# Autodesk Inventor assembly: Sostenedor puerta caja
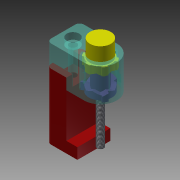
[picture p0: Inventor's stored thumbnail of the model, 180x180]
Saved by Autodesk Inventor 2014 (Build 180170000, 170)
## iProperties
Created: 2017-02-07
Part Number: Sostenedor puerta caja
Document SubType Name: Assembly
Designer: Rubén
Author: Rubén
## Documents named in this file (6)
- C:\Users\Rubén\Desktop\Mis diseños\Sostenedor puerta caja\src\Assembly.iam
- C:\Users\Rubén\Desktop\Mis diseños\Sostenedor puerta caja\src\Case (part 1).ipt
- C:\Users\Rubén\Desktop\Mis diseños\Sostenedor puerta caja\src\Case (part 2).ipt
- C:\Users\Rubén\Desktop\Mis diseños\Sostenedor puerta caja\src\Button.ipt
- C:\Users\Rubén\Desktop\Mis diseños\Sostenedor puerta caja\src\Rotor.ipt
- C:\Users\Rubén\Desktop\Mis diseños\Sostenedor puerta caja\src\Screw.ipt
## Components (5 placed, 5 different names)
1. Case (part 1):1 — Mate:1, Mate:2, Angle:1, Mate:3, Angle:2, Flush:2, Angle:3, Mate:8
2. Case (part 2):1 — Mate:1, Mate:2, Angle:1
3. Button:1 — Mate:3, Angle:2, Mate:4, Mate:5, Mate:8
4. Rotor:1 — Mate:4, Flush:2, Angle:3, Mate:5, Mate:6, Mate:7
5. Screw:1 — Mate:6, Mate:7
## Relationships (12: Mate 8, Angle 3, Flush 1)
- Mate:1: Case (part 1):1 ↔ Case (part 2):1
- Mate:2: Case (part 1):1 ↔ Case (part 2):1
- Angle:1 (0 deg): Case (part 1):1 ↔ Case (part 2):1
- Mate:3: Case (part 1):1 ↔ Button:1
- Angle:2 (0 deg): Case (part 1):1 ↔ Button:1
- Mate:4: Button:1 ↔ Rotor:1
- Flush:2: Case (part 1):1 ↔ Rotor:1
- Angle:3 (0 deg): Case (part 1):1 ↔ Rotor:1
- Mate:5: Button:1 ↔ Rotor:1
- Mate:6: Rotor:1 ↔ Screw:1
- Mate:7: Rotor:1 ↔ Screw:1
- Mate:8: Case (part 1):1 ↔ Button:1
